# Autodesk Inventor assembly: Chessboard Design
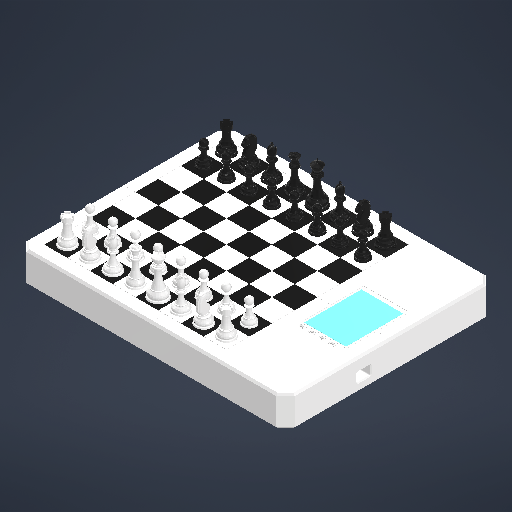
[picture p0: Inventor's stored thumbnail of the model, 512x512]
Saved by Autodesk Inventor 2026 (Build 300175000, 175)
## iProperties
Created: 2025-06-07
Part Number: Chessboard Design
Document SubType Name: Assembly
Designer: ckyiu
Author: ckyiu
## Documents named in this file (4)
- F:\Chessboard-Design\Assemblies\Chessboard Design.iam
- F:\Chessboard-Design\Assemblies\Chessboard Design Core.iam
- F:\Chessboard-Design\Assemblies\Case\Case Bottom.iam
- F:\Chessboard-Design\Parts\Case\Case Top.ipt
## Components (3 placed, 3 different names)
1. Case Bottom:1 [sub-assembly] — Insert:1, Angle:1, Mate:1, Mate:2, Mate:3
2. Chessboard Design Core:1 [sub-assembly] — Insert:1, Angle:1
3. Case Top:1 — Mate:1, Mate:2, Mate:3
## Relationships (5: Mate 3, Insert 1, Angle 1)
- Insert:1: Case Bottom:1 ↔ Chessboard Design Core:1
- Angle:1 (0 deg): Case Bottom:1 ↔ Chessboard Design Core:1
- Mate:1: Case Bottom:1 ↔ Case Top:1
- Mate:2: Case Bottom:1 ↔ Case Top:1
- Mate:3: Case Bottom:1 ↔ Case Top:1
